# Autodesk Inventor assembly: PEG
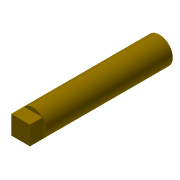
[picture p0: Inventor's stored thumbnail of the model, 180x180]
Saved by Autodesk Inventor 2015 (Build 190159000, 159)
## iProperties
Created: 2015-03-07
Part Number: PEG
Document SubType Name: Assembly
Designer: Jaden
Author: Jaden
## Documents named in this file (3)
- E:\ReDesign\PEG.iam
- E:\ReDesign\Peg.ipt
- E:\ReDesign\PegHead.ipt
## Components (2 placed, 2 different names)
1. Peg:1 — Mate:1, Tangent:1
2. PegHead:1 — Mate:1, Tangent:1
## Relationships (2: Mate 1, Tangent 1)
- Mate:1: Peg:1 ↔ PegHead:1
- Tangent:1: Peg:1 ↔ PegHead:1
